# Autodesk Inventor assembly: 6P Sprocket
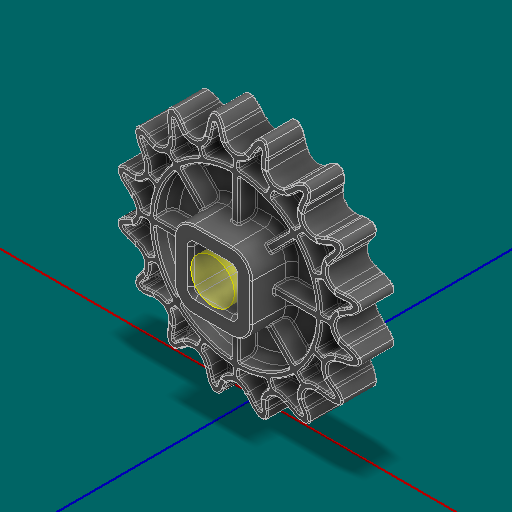
[picture p0: Inventor's stored thumbnail of the model, 512x512]
Saved by Autodesk Inventor 2025 (Build 290162000, 162)
## iProperties
Created: 2022-08-02
Part Number: 6P Sprocket
Document SubType Name: Assembly
Designer: ylu12
Author: ylu12
## Documents named in this file (23)
- C:\Users\avere\VEX\High Stakes\CAD\ROBOPROS-CAD-Inventor\Motion\Sprockets\6P Sprocket.iam
- C:\Users\avere\VEX\High Stakes\CAD\ROBOPROS-CAD-Inventor\Motion\HS Shaft Adapter Circle.ipt
- C:\Users\avere\VEX\High Stakes\CAD\ROBOPROS-CAD-Inventor\Motion\HS Shaft Adapter Square.ipt
- C:\Users\avere\VEX\High Stakes\CAD\ROBOPROS-CAD-Inventor\Motion\Sprockets\Reference Files\6P 8T Sprocket.ipt
- C:\Users\avere\VEX\High Stakes\CAD\ROBOPROS-CAD-Inventor\Motion\Sprockets\Reference Files\6P 16T Sprocket.ipt
- C:\Users\avere\VEX\High Stakes\CAD\ROBOPROS-CAD-Inventor\Motion\Sprockets\Reference Files\6P 24T Sprocket.ipt
- C:\Users\avere\VEX\High Stakes\CAD\ROBOPROS-CAD-Inventor\Motion\Sprockets\Reference Files\6P 32T Sprocket.ipt
- C:\Users\avere\VEX\High Stakes\CAD\ROBOPROS-CAD-Inventor\Motion\Sprockets\Reference Files\6P 40T Sprocket.ipt
- 6P 16T Sprocket, Circle.iam
- 6P 16T Sprocket, No Insert.iam
- 6P 16T Sprocket, Square.iam
- 6P 24T Sprocket, Circle.iam
- 6P 24T Sprocket, No Insert.iam
- 6P 24T Sprocket, Square.iam
- 6P 32T Sprocket, Circle.iam
- 6P 32T Sprocket, No Insert.iam
- 6P 32T Sprocket, Square.iam
- 6P 40T Sprocket, Circle.iam
- 6P 40T Sprocket, No Insert.iam
- 6P 40T Sprocket, Square.iam
- 6P 8T Sprocket, Circle.iam
- 6P 8T Sprocket, No Insert.iam
- 6P 8T Sprocket, Square.iam
## Components (7 placed, 7 different names)
1. Circle — Flush:1, Mate:1, Mate:3
2. Square — Flush:2, Mate:2, Mate:4
3. 8T — Mate:5, Mate:6, Flush:3
4. 16T — Flush:4, Mate:7, Mate:8
5. 24T — Flush:5, Mate:9, Mate:10
6. 32T — Flush:6, Mate:11, Mate:12
7. 40T — Flush:7, Mate:13, Mate:14
## Relationships (21: Mate 14, Flush 7)
- Flush:1 (6.35 mm): Circle
- Flush:2 (6.35 mm): Square
- Mate:1: Circle
- Mate:2: Square
- Mate:3: Circle
- Mate:4: Square
- Mate:5: 8T
- Mate:6: 8T
- Flush:3: 8T
- Flush:4: 16T
- Flush:5: 24T
- Flush:6: 32T
- Flush:7: 40T
- Mate:7: 16T
- Mate:8: 16T
- Mate:9: 24T
- Mate:10: 24T
- Mate:11: 32T
- Mate:12: 32T
- Mate:13: 40T
- Mate:14: 40T
